# Autodesk Inventor assembly: FinalAssembly
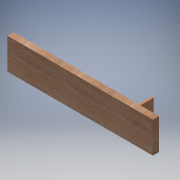
[picture p0: Inventor's stored thumbnail of the model, 180x180]
Saved by Autodesk Inventor 2018 (Build 220112000, 112)
## iProperties
Created: 2019-05-10
Part Number: FinalAssembly
Document SubType Name: Assembly
Designer: aal_9
Author: aal_9
## Documents named in this file (10)
- C:\Users\aal_9\OneDrive\Documentos\Suiza\Courses\Tesis\TestBench\FinalAssembly.iam
- C:\Users\aal_9\OneDrive\Documentos\Suiza\Courses\Tesis\TestBench\Base.ipt
- C:\Users\aal_9\OneDrive\Documentos\Suiza\Courses\Tesis\TestBench\SupportCylinder.ipt
- C:\Users\aal_9\OneDrive\Documentos\Suiza\Courses\Tesis\TestBench\AIS2017\19197 DSNU-12-200-P-A---(0).iam
- C:\Users\aal_9\OneDrive\Documentos\Suiza\Courses\Tesis\TestBench\Force_Sensor.ipt
- C:\Users\aal_9\OneDrive\Documentos\Suiza\Courses\Tesis\TestBench\CopleCylinderSensor.ipt
- C:\Users\aal_9\OneDrive\Documentos\Suiza\Courses\Tesis\TestBench\CopleCatheter.ipt
- C:\Users\aal_9\OneDrive\Documentos\Suiza\Courses\Tesis\TestBench\cathetherEntry.ipt
- C:\Users\aal_9\OneDrive\Documentos\Suiza\Courses\Tesis\TestBench\FinalAssembly\Design Accelerator\Compress Spring2.iam
- C:\Users\aal_9\OneDrive\Documentos\Suiza\Courses\Tesis\TestBench\Nut.ipt
## Components (10 placed, 9 different names)
1. Base:1 — Mate:1, Mate:2, Mate:3, Mate:4, Mate:5, Mate:6, Mate:14, Flush:1, Mate:15
2. SupportCylinder:1 — Mate:4, Mate:5, Mate:6, Cylindrical:1
3. SupportCylinder:2 — Mate:1, Mate:2, Mate:3, Mate:7
4. 19197 DSNU-12-200-P-A---(0):1 [sub-assembly] — Mate:7, Cylindrical:1, Mate:8, Mate:9, Mate:16
5. Force_Sensor:1 — Mate:10, Mate:11, Mate:12, Mate:13
6. CopleCylinderSensor:1 — Mate:8, Mate:9, Mate:10, Mate:11, Mate:17, Mate:18
7. CopleCatheter:1 — Mate:12, Mate:13
8. cathetherEntry:1 — Mate:14, Flush:1, Mate:15
9. Compress Spring:1 [sub-assembly] — Mate:16
10. Nut:1 — Mate:17, Mate:18
## Relationships (20: Mate 18, CylindricalJoint 1, Flush 1)
- Mate:1: Base:1 ↔ SupportCylinder:2
- Mate:2: Base:1 ↔ SupportCylinder:2
- Mate:3: Base:1 ↔ SupportCylinder:2
- Mate:4: Base:1 ↔ SupportCylinder:1
- Mate:5: Base:1 ↔ SupportCylinder:1
- Mate:6: Base:1 ↔ SupportCylinder:1
- Mate:7: SupportCylinder:2 ↔ 19197 DSNU-12-200-P-A---(0):1
- Cylindrical:1: SupportCylinder:1 ↔ 19197 DSNU-12-200-P-A---(0):1
- Mate:8: 19197 DSNU-12-200-P-A---(0):1 ↔ CopleCylinderSensor:1
- Mate:9: 19197 DSNU-12-200-P-A---(0):1 ↔ CopleCylinderSensor:1
- Mate:10: Force_Sensor:1 ↔ CopleCylinderSensor:1
- Mate:11: Force_Sensor:1 ↔ CopleCylinderSensor:1
- Mate:12: Force_Sensor:1 ↔ CopleCatheter:1
- Mate:13 (-4 mm): Force_Sensor:1 ↔ CopleCatheter:1
- Mate:14: Base:1 ↔ cathetherEntry:1
- Flush:1: Base:1 ↔ cathetherEntry:1
- Mate:15: Base:1 ↔ cathetherEntry:1
- Mate:16: 19197 DSNU-12-200-P-A---(0):1 ↔ Compress Spring:1
- Mate:17: CopleCylinderSensor:1 ↔ Nut:1
- Mate:18: CopleCylinderSensor:1 ↔ Nut:1
